# Autodesk Inventor assembly: HM1_FIXT1_CAM1
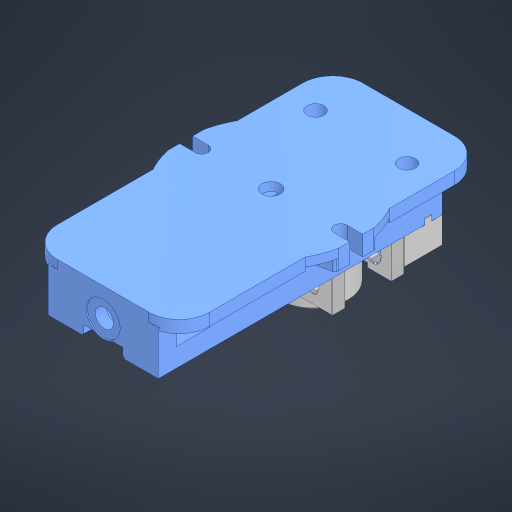
[picture p0: Inventor's stored thumbnail of the model, 512x512]
Saved by Autodesk Inventor 2024.3 (Build 283343000, 343)
## iProperties
Created: 2024-08-20
Part Number: HM1_FIXT1_CAM1
Document SubType Name: Assembly
Designer: fablabadmin
Author: fablabadmin
## Documents named in this file (8)
- C:\Users\fablabadmin\Documents\_Benjamin_S\_3dCAD\HHVerkstad\Hammer\_FIXT\_FIXT1-001_CAM1\HM1_FIXT1-001_CAM1.iam
- C:\Users\fablabadmin\Documents\_Benjamin_S\_3dCAD\_Config\KemmlerVise\OP1-KemmlerVise.iam
- C:\Users\fablabadmin\Documents\_Benjamin_S\_3dCAD\_Config\KemmlerVise\OP2-KemmlerVise.iam
- C:\Users\fablabadmin\Documents\_Benjamin_S\_3dCAD\HHVerkstad\Hammer\_FIXT\HM1_FIXT1-001.ipt
- C:\Users\fablabadmin\Documents\_Benjamin_S\_3dCAD\HHVerkstad\Hammer\_FIXT\_FIXT1-001_CAM1\JawDualSided-Aluminum 6061.ipt
- C:\Users\fablabadmin\Documents\_Benjamin_S\_3dCAD\HHVerkstad\Hammer\_FIXT\_FIXT1-001_CAM1\RoundStock.ipt
- C:\Users\fablabadmin\Documents\_Benjamin_S\_3dCAD\HHVerkstad\Hammer\_FIXT\_FIXT1-001_CAM1\JawDualSided-Aluminum 6061MIR.ipt
- C:\Users\fablabadmin\Documents\_Benjamin_S\_3dCAD\_Config\_CAM_SIM\FixtureParts\parallels3mm.xlsx
## Components (8 placed, 6 different names)
1. HM1_FIXT1-001:1 — Mate:3, Flush:2, Mate:9, Tangent:5, Tangent:6, Tangent:7, Mate:10
2. RoundStock:1 — Mate:3, Flush:2, Tangent:1, Tangent:2, Mate:4, Tangent:3, Tangent:4
3. OP1-KemmlerVise:1 [sub-assembly] — Mate:1, Flush:1, Mate:2, Mate:5, Angle:1, Angle:2
4. JawDualSided-Aluminum 6061:1 — Mate:1, Flush:1, Mate:2, Tangent:1, Tangent:2, Mate:4, Flush:3
5. JawDualSided-Aluminum 6061MIR:1 — Mate:5, Flush:3, Tangent:3, Tangent:4
6. OP2-KemmlerVise:1 [sub-assembly] — Mate:6, Mate:7, Flush:4, Mate:8, Angle:2, Mate:11
7. JawDualSided-Aluminum 6061:2 — Mate:6, Flush:4, Flush:5, Mate:8, Mate:9, Tangent:5, Tangent:6
8. JawDualSided-Aluminum 6061MIR:2 — Mate:7, Flush:5, Tangent:7
## Relationships (26: Mate 12, Tangent 7, Flush 5, Angle 2)
- Mate:1: OP1-KemmlerVise:1 ↔ JawDualSided-Aluminum 6061:1
- Flush:1: OP1-KemmlerVise:1 ↔ JawDualSided-Aluminum 6061:1
- Mate:2: OP1-KemmlerVise:1 ↔ JawDualSided-Aluminum 6061:1
- Mate:3: HM1_FIXT1-001:1 ↔ RoundStock:1
- Flush:2 (-7 mm): HM1_FIXT1-001:1 ↔ RoundStock:1
- Tangent:1: RoundStock:1 ↔ JawDualSided-Aluminum 6061:1
- Tangent:2: RoundStock:1 ↔ JawDualSided-Aluminum 6061:1
- Mate:4: RoundStock:1 ↔ JawDualSided-Aluminum 6061:1
- Mate:5: OP1-KemmlerVise:1 ↔ JawDualSided-Aluminum 6061MIR:1
- Flush:3: JawDualSided-Aluminum 6061:1 ↔ JawDualSided-Aluminum 6061MIR:1
- Tangent:3: RoundStock:1 ↔ JawDualSided-Aluminum 6061MIR:1
- Tangent:4: RoundStock:1 ↔ JawDualSided-Aluminum 6061MIR:1
- Mate:6: OP2-KemmlerVise:1 ↔ JawDualSided-Aluminum 6061:2
- Mate:7: OP2-KemmlerVise:1 ↔ JawDualSided-Aluminum 6061MIR:2
- Flush:4: OP2-KemmlerVise:1 ↔ JawDualSided-Aluminum 6061:2
- Flush:5: JawDualSided-Aluminum 6061:2 ↔ JawDualSided-Aluminum 6061MIR:2
- Mate:8: OP2-KemmlerVise:1 ↔ JawDualSided-Aluminum 6061:2
- Mate:9: HM1_FIXT1-001:1 ↔ JawDualSided-Aluminum 6061:2
- Tangent:5: HM1_FIXT1-001:1 ↔ JawDualSided-Aluminum 6061:2
- Tangent:6: HM1_FIXT1-001:1 ↔ JawDualSided-Aluminum 6061:2
- Tangent:7: HM1_FIXT1-001:1 ↔ JawDualSided-Aluminum 6061MIR:2
- Angle:1 (0 deg): OP1-KemmlerVise:1
- Angle:2 (0 deg): OP1-KemmlerVise:1 ↔ OP2-KemmlerVise:1
- Mate:10: HM1_FIXT1-001:1
- Mate:11: OP2-KemmlerVise:1
- Mate:12
## Named parameters: PRL13 = 13 mm, PRL16 = 16 mm, PRL19 = 19 mm, PRL22 = 22 mm, PRL28 = 28 mm, PRL31 = 31 mm, PRL35 = 35 mm, PRL38 = 38 mm, PRL41 = 41 mm
